# Autodesk Inventor assembly: sprezyna49_final
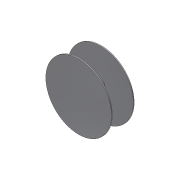
[picture p0: Inventor's stored thumbnail of the model, 180x180]
Saved by Autodesk Inventor 2017 (Build 210142000, 142)
## iProperties
Created: 2018-03-07
Part Number: sprezyna49_final
Document SubType Name: Assembly
Designer: Dazzyl
Author: Dazzyl
## Documents named in this file (3)
- C:\Users\Dazzyl\Desktop\sprezyna49_final.iam
- C:\Users\Dazzyl\Desktop\sprezyna49_final\Design Accelerator\Sprężyna naciskowa1.iam
- C:\Users\Dazzyl\Desktop\plate_beta.ipt
## Components (3 placed, 2 different names)
1. Sprężyna naciskowa:1 [sub-assembly] — Zestawiający:1, Zestawiający:2, Zestawiający:3, Zestawiający:4
2. plate_beta:1 — Zestawiający:3, Zestawiający:5
3. plate_beta:2 — Zestawiający:4, Zestawiający:5
## Relationships (5: Mate 5)
- Zestawiający:1 [Mate]: Sprężyna naciskowa:1
- Zestawiający:2 [Mate]: Sprężyna naciskowa:1
- Zestawiający:3 [Mate]: Sprężyna naciskowa:1 ↔ plate_beta:1
- Zestawiający:4 [Mate]: Sprężyna naciskowa:1 ↔ plate_beta:2
- Zestawiający:5 [Mate]: plate_beta:1 ↔ plate_beta:2
